# Autodesk Inventor assembly: Robot
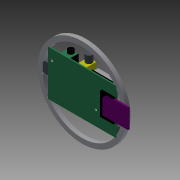
[picture p0: Inventor's stored thumbnail of the model, 180x180]
Saved by Autodesk Inventor 2014 (Build 180170000, 170)
## iProperties
Created: 2013-05-24
Part Number: Robot
Document SubType Name: Assembly
Designer: hartmann
Author: hartmann
## Documents named in this file (3)
- C:\Dokumente und Einstellungen\hartmann\Desktop\Robot\Robot.iam
- C:\Dokumente und Einstellungen\hartmann\Desktop\RaspberryPi\RaspberryPi.iam
- C:\Dokumente und Einstellungen\hartmann\Desktop\Robot\frame.ipt
## Components (2 placed, 2 different names)
1. RaspberryPi:1 [sub-assembly] — Fluchtend:1
2. frame:1 — Fluchtend:1
## Relationships (1: Flush 1)
- Fluchtend:1 [Flush]: RaspberryPi:1 ↔ frame:1
